# Autodesk Inventor assembly: Link1
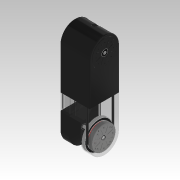
[picture p0: Inventor's stored thumbnail of the model, 180x180]
Saved by Autodesk Inventor 2020 (Build 240168000, 168)
## iProperties
Created: 2021-11-21
Part Number: Link1
Document SubType Name: Assembly
Designer: DDeGo
Author: DDeGo
## Documents named in this file (15)
- C:\Users\DDeGo\Documents\Drew\Projects\OS-ARM\cad\FirstDraft\Link1.iam
- C:\Users\DDeGo\Documents\Drew\Projects\OS-ARM\cad\FirstDraft\Link1a.ipt
- C:\Users\DDeGo\Documents\Drew\Projects\OS-ARM\cad\FirstDraft\Link1b.ipt
- C:\Users\DDeGo\Documents\Drew\Projects\OS-ARM\cad\OTS\Electronics\NEMA 23 - 41mm.ipt
- C:\Users\DDeGo\Documents\Drew\Projects\OS-ARM\cad\HarmonicDrive75mm V2\HarmonicDrive75mmV2.iam
- C:\Users\DDeGo\Documents\Drew\Projects\OS-ARM\cad\OTS\Radial Bearings\6815 bearing.ipt
- C:\Users\DDeGo\Documents\Drew\Projects\OS-ARM\cad\OTS\Other\M8x85mm Threaded Rod.ipt
- C:\Users\DDeGo\Documents\Drew\Projects\OS-ARM\cad\OTS\Other\CF Tube 6x4x250.ipt
- C:\Users\DDeGo\Documents\Drew\Projects\OS-ARM\cad\OTS\Other\CF Tube 4x2x100.ipt
- C:\Users\DDeGo\Documents\Drew\Projects\OS-ARM\cad\OTS\Other\GT2 20T Drive Pulley.ipt
- C:\Users\DDeGo\Documents\Drew\Projects\OS-ARM\cad\FirstDraft\J2MotorBracket.ipt
- C:\Users\DDeGo\Documents\Drew\Projects\OS-ARM\cad\OTS\Other\GT2 60T Drive Pulley.ipt
- C:\Users\DDeGo\Documents\Drew\Projects\OS-ARM\cad\OTS\Radial Bearings\688 bearing.ipt
- C:\Users\DDeGo\Documents\Drew\Projects\OS-ARM\cad\OTS\Radial Bearings\608 bearing.ipt
- C:\Users\DDeGo\Documents\Drew\Projects\OS-ARM\cad\FirstDraft\Link1c.ipt
## Components (22 placed, 14 different names)
1. Link1a:1 — Mate:1, Flush:1, Mate:2, Mate:3, Mate:4, Mate:10, Mate:23, Mate:24, Mate:25, Mate:34, Mate:35, Mate:36, Mate:37, Mate:38, Mate:39, Mate:40, Mate:41
2. Link1b:1 — Mate:3, Mate:4, Mate:9, Mate:10, Mate:11, Mate:12, Mate:14, Mate:15, Mate:16, Mate:17, Mate:18, Mate:19, Mate:20, Mate:21, Mate:22, Mate:44, Mate:45, Flush:11, Flush:12
3. NEMA 23 - 41mm:1 — Mate:26, Mate:27, Mate:28, Mate:29, Mate:30
4. HarmonicDrive75mmV2:1 [sub-assembly] — Mate:6, Mate:7, Mate:11, Mate:12, Flush:2, Flush:9, Mate:42
5. 6815 bearing:1 — Mate:6, Mate:7, Mate:9
6. M8x85mm Threaded Rod:1 — Flush:2, Mate:31, Flush:9, Flush:10, Mate:42, Mate:43
7. CF Tube 6x4x250:1 — Mate:15, Flush:7
8. CF Tube 4x2x100:1 — Flush:3, Mate:18
9. CF Tube 6x4x250:2 — Mate:14, Flush:7, Mate:22
10. CF Tube 4x2x100:2 — Flush:6, Mate:16
11. CF Tube 4x2x100:3 — Flush:5, Mate:19
12. CF Tube 4x2x100:4 — Flush:4, Mate:17
13. CF Tube 4x2x100:5 — Flush:3, Flush:4, Flush:5, Flush:6, Mate:20, Mate:21
14. GT2 20T Drive Pulley:1 — Mate:29, Mate:30, Flush:8
15. J2MotorBracket:1 — Mate:23, Mate:24, Mate:25, Mate:26, Mate:27, Mate:28
16. GT2 60T Drive Pulley:1 — Mate:31, Flush:8, Flush:10
17. 688 bearing:1 — Mate:43, Mate:46
18. 608 bearing:1 — Mate:36, Mate:41
19. 608 bearing:2 — Mate:37, Mate:38
20. 688 bearing:2 — Mate:34, Mate:40
21. 688 bearing:3 — Mate:35, Mate:39
22. Link1c:1 — Mate:44, Mate:45, Flush:11, Flush:12, Mate:46
## Relationships (53: Mate 41, Flush 12)
- Mate:1: Link1a:1
- Flush:1: Link1a:1
- Mate:2: Link1a:1
- Mate:3: Link1a:1 ↔ Link1b:1
- Mate:4: Link1a:1 ↔ Link1b:1
- Mate:6: HarmonicDrive75mmV2:1 ↔ 6815 bearing:1
- Mate:7: HarmonicDrive75mmV2:1 ↔ 6815 bearing:1
- Mate:9: Link1b:1 ↔ 6815 bearing:1
- Mate:10: Link1a:1 ↔ Link1b:1
- Mate:11: Link1b:1 ↔ HarmonicDrive75mmV2:1
- Mate:12: Link1b:1 ↔ HarmonicDrive75mmV2:1
- Flush:2 (1 mm): HarmonicDrive75mmV2:1 ↔ M8x85mm Threaded Rod:1
- Mate:14: Link1b:1 ↔ CF Tube 6x4x250:2
- Mate:15: Link1b:1 ↔ CF Tube 6x4x250:1
- Flush:3: CF Tube 4x2x100:1 ↔ CF Tube 4x2x100:5
- Flush:4: CF Tube 4x2x100:4 ↔ CF Tube 4x2x100:5
- Flush:5: CF Tube 4x2x100:3 ↔ CF Tube 4x2x100:5
- Flush:6: CF Tube 4x2x100:2 ↔ CF Tube 4x2x100:5
- Mate:16: Link1b:1 ↔ CF Tube 4x2x100:2
- Mate:17: Link1b:1 ↔ CF Tube 4x2x100:4
- Mate:18: Link1b:1 ↔ CF Tube 4x2x100:1
- Mate:19: Link1b:1 ↔ CF Tube 4x2x100:3
- Mate:20: Link1b:1 ↔ CF Tube 4x2x100:5
- Mate:21 (2 mm): Link1b:1 ↔ CF Tube 4x2x100:5
- Flush:7: CF Tube 6x4x250:1 ↔ CF Tube 6x4x250:2
- Mate:22 (2 mm): Link1b:1 ↔ CF Tube 6x4x250:2
- Mate:23: Link1a:1 ↔ J2MotorBracket:1
- Mate:24: Link1a:1 ↔ J2MotorBracket:1
- Mate:25: Link1a:1 ↔ J2MotorBracket:1
- Mate:26: NEMA 23 - 41mm:1 ↔ J2MotorBracket:1
- Mate:27: NEMA 23 - 41mm:1 ↔ J2MotorBracket:1
- Mate:28: NEMA 23 - 41mm:1 ↔ J2MotorBracket:1
- Mate:29: NEMA 23 - 41mm:1 ↔ GT2 20T Drive Pulley:1
- Mate:30 (5 mm): NEMA 23 - 41mm:1 ↔ GT2 20T Drive Pulley:1
- Mate:31: M8x85mm Threaded Rod:1 ↔ GT2 60T Drive Pulley:1
- Flush:8: GT2 20T Drive Pulley:1 ↔ GT2 60T Drive Pulley:1
- Flush:9: HarmonicDrive75mmV2:1 ↔ M8x85mm Threaded Rod:1
- Flush:10: M8x85mm Threaded Rod:1 ↔ GT2 60T Drive Pulley:1
- Mate:34: Link1a:1 ↔ 688 bearing:2
- Mate:35: Link1a:1 ↔ 688 bearing:3
- Mate:36: Link1a:1 ↔ 608 bearing:1
- Mate:37: Link1a:1 ↔ 608 bearing:2
- Mate:38: Link1a:1 ↔ 608 bearing:2
- Mate:39: Link1a:1 ↔ 688 bearing:3
- Mate:40: Link1a:1 ↔ 688 bearing:2
- Mate:41: Link1a:1 ↔ 608 bearing:1
- Mate:42: HarmonicDrive75mmV2:1 ↔ M8x85mm Threaded Rod:1
- Mate:43: M8x85mm Threaded Rod:1 ↔ 688 bearing:1
- Mate:44: Link1b:1 ↔ Link1c:1
- Mate:45: Link1b:1 ↔ Link1c:1
- Flush:11: Link1b:1 ↔ Link1c:1
- Flush:12: Link1b:1 ↔ Link1c:1
- Mate:46: 688 bearing:1 ↔ Link1c:1
